# Autodesk Inventor assembly: thumb_plate
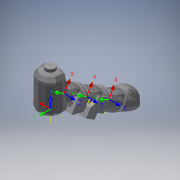
[picture p0: Inventor's stored thumbnail of the model, 180x180]
Saved by Autodesk Inventor 2019 (Build 230136000, 136)
## iProperties
Created: 2024-08-27
Part Number: thumb_plate
Material: Generisch
Document SubType Name: Assembly
Designer: nic
Author: nic
## Documents named in this file (4)
- C:\Users\Nicolas Frick\Sync\OneDrive\wtm\nicol_rh8d\inventor\thumb_plate.iam
- C:\Users\Nicolas Frick\Sync\OneDrive\wtm\nias\nias_description\inventor_files\hand\r_rh8d_refac\thumb base refac.iam
- C:\Users\Nicolas Frick\Sync\OneDrive\wtm\nicol_rh8d\inventor\thumb_base_plate.ipt
- C:\Users\Nicolas Frick\Sync\OneDrive\wtm\nicol_rh8d\inventor\thumb_phalanx_plate.ipt
## Components (3 placed, 3 different names)
1. thumb base refac:1 [sub-assembly] — Passend:1, Passend:2, Fluchtend:1, Fluchtend:2
2. thumb_base_plate:1 — Fluchtend:2, Fluchtend:3
3. thumb_phalanx_plate:1 — Fluchtend:3
## Relationships (5: Flush 3, Mate 2)
- Passend:1 [Mate]: thumb base refac:1
- Passend:2 [Mate]: thumb base refac:1
- Fluchtend:1 [Flush]: thumb base refac:1
- Fluchtend:2 [Flush]: thumb base refac:1 ↔ thumb_base_plate:1
- Fluchtend:3 [Flush]: thumb_base_plate:1 ↔ thumb_phalanx_plate:1
